# Autodesk Inventor assembly: cover_final_assembly
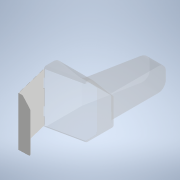
[picture p0: Inventor's stored thumbnail of the model, 180x180]
Saved by Autodesk Inventor 2021 (Build 250183000, 183)
## iProperties
Created: 2021-06-25
Part Number: cover_final_assembly
Document SubType Name: Assembly
## Documents named in this file (3)
- C:\Users\ocon0143\OneDrive - Flinders\Advn Mech Design Shared\6_Development\2_Design\inventor\cover\cover_final_assembly.iam
- C:\Users\ocon0143\OneDrive - Flinders\Advn Mech Design Shared\6_Development\2_Design\inventor\vehicle_wheelchair\wheelchair\wheelchair_box_extended.ipt
- C:\Users\ocon0143\OneDrive - Flinders\Advn Mech Design Shared\6_Development\2_Design\inventor\cover\cover_open_door.ipt
## Components (2 placed, 2 different names)
1. wheelchair_box_extended:1 — Mate:1, Flush:1, Flush:2, Mate:2, Flush:3
2. cover_open_door:1 — Mate:2, Flush:3
## Relationships (5: Flush 3, Mate 2)
- Mate:1: wheelchair_box_extended:1
- Flush:1: wheelchair_box_extended:1
- Flush:2: wheelchair_box_extended:1
- Mate:2: wheelchair_box_extended:1 ↔ cover_open_door:1
- Flush:3 (50 mm): wheelchair_box_extended:1 ↔ cover_open_door:1
